# Autodesk Inventor assembly: ASY NDM 4.0 домкрат
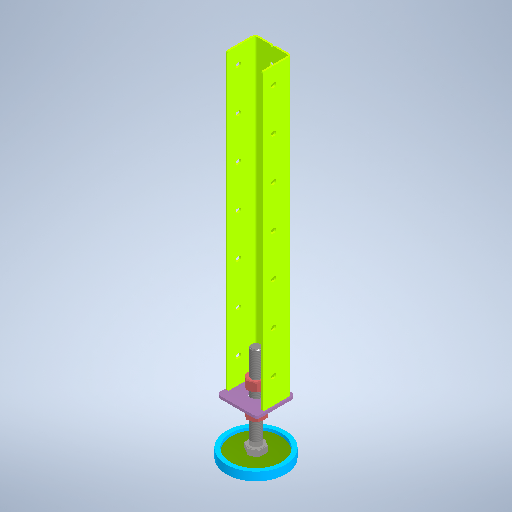
[picture p0: Inventor's stored thumbnail of the model, 512x512]
Saved by Autodesk Inventor 2025 (Build 290162010, 162A)
## iProperties
Created: 2023-07-06
Part Number: ASY NDM 4.0 домкрат
Document SubType Name: Assembly
Designer: user
Stock Number: NDM 4.0 домкрат
Description: сборочная ед.
Author: user
Revision Number: 1
## Documents named in this file (8)
- C:\Users\admin\YandexDisk-badmisterfox\домашниий пк\Inventor\Nadyim\CAD\Screwjack pilar\ASY NDM 14.0 Screwjack pillar 1.iam
- C:\Users\admin\YandexDisk-badmisterfox\домашниий пк\Inventor\Nadyim\CAD\NDM 7.1 bracket bottom father.ipt
- C:\Users\admin\YandexDisk-badmisterfox\домашниий пк\Inventor\Nadyim\CAD\Screwjack pilar\NDM 12.2 square plate.ipt
- C:\Users\admin\YandexDisk-badmisterfox\домашниий пк\Inventor\Nadyim\CAD\Screwjack pilar\NDM 14.1  plastic plate.ipt
- C:\Users\admin\YandexDisk-badmisterfox\домашниий пк\Inventor\Nadyim\CAD\Screwjack pilar\NDM 12.1 base plate.ipt
- C:\Users\admin\YandexDisk-badmisterfox\домашниий пк\Inventor\Nadyim\Content Center Files\en-US\DIN EN ISO 4017\DIN EN ISO 4017 - M12 x 100.ipt
- C:\Users\admin\YandexDisk-badmisterfox\домашниий пк\Inventor\Nadyim\CAD\NMD 23 Опорный кронштейн.ipt
- C:\Users\admin\YandexDisk-badmisterfox\домашниий пк\Inventor\Nadyim\Content Center Files\en-US\Гайка SS ISO 4032\Copy of ISO 4032 - M12 - ISO.ipt
## Components (8 placed, 7 different names)
1. NDM 7.1 bracket bottom father:1 — Flush:1, Mate:1, Mate:2, Flush:3, Flush:4
2. NDM 12.2 square plate:1 — Mate:2, Flush:3, Flush:4, Rigid:10
3. DIN EN ISO 4017 M12 x 100:1 — Rigid:6, Cylindrical:1, Cylindrical:2
4. NDM 14.1  plastic plate:1 — Rigid:9, Mate:3, Rigid:10
5. NDM 12.1 base plate:1 — Rigid:6, Rigid:9
6. NMD 23 Опорный кронштейн:1
7. Гайка SS ISO 4032 M12:2 — Cylindrical:1
8. Гайка SS ISO 4032 M12:3 — Cylindrical:2
## Relationships (11: Flush 3, Mate 3, WeldJoint 3, CylindricalJoint 2)
- Flush:1: NDM 7.1 bracket bottom father:1
- Mate:1 (22 mm): NDM 7.1 bracket bottom father:1
- Rigid:6 [WeldJoint]: DIN EN ISO 4017 M12 x 100:1 ↔ NDM 12.1 base plate:1
- Mate:2: NDM 7.1 bracket bottom father:1 ↔ NDM 12.2 square plate:1
- Flush:3 (-2 mm): NDM 7.1 bracket bottom father:1 ↔ NDM 12.2 square plate:1
- Flush:4 (-2 mm): NDM 7.1 bracket bottom father:1 ↔ NDM 12.2 square plate:1
- Rigid:9 [WeldJoint]: NDM 14.1  plastic plate:1 ↔ NDM 12.1 base plate:1
- Mate:3: NDM 14.1  plastic plate:1
- Rigid:10 [WeldJoint] (62 mm): NDM 12.2 square plate:1 ↔ NDM 14.1  plastic plate:1
- Cylindrical:1: DIN EN ISO 4017 M12 x 100:1 ↔ Гайка SS ISO 4032 M12:2
- Cylindrical:2: DIN EN ISO 4017 M12 x 100:1 ↔ Гайка SS ISO 4032 M12:3
